# Autodesk Inventor assembly: platform
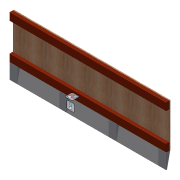
[picture p0: Inventor's stored thumbnail of the model, 180x180]
Saved by Autodesk Inventor 2015 (Build 190159000, 159)
## iProperties
Created: 2015-01-03
Part Number: platform
Document SubType Name: Assembly
Designer: Peter
Mass: 10587 g
Surface Area: 19021.5 cm^2
Volume: 16103.8 cm^3
Density: 0.657427 g/cm^3
Author: Peter
## Documents named in this file (5)
- T:\FILES\FIRST-Team-1719-CAD-Team\2015 Playing Field\Team 1719 Practice Field\Scoring Platform - Construction Design\platform.iam
- T:\FILES\FIRST-Team-1719-CAD-Team\2015 Playing Field\Team 1719 Practice Field\Scoring Platform - Construction Design\plywood platform.ipt
- T:\FILES\FIRST-Team-1719-CAD-Team\2015 Playing Field\Team 1719 Practice Field\Scoring Platform - Construction Design\2x4x48.ipt
- T:\FILES\FIRST-Team-1719-CAD-Team\2015 Playing Field\Team 1719 Practice Field\Scoring Platform - Construction Design\Ramp Assembly.iam
- T:\FILES\FIRST-Team-1719-CAD-Team\2015 Playing Field\Team 1719 Practice Field\Scoring Platform - Construction Design\Wedge.ipt
## Components (8 placed, 4 different names)
1. plywood platform:1 — Mate:1, Flush:1, Flush:2, Flush:3, Flush:4, Mate:2, Mate:3, Flush:5
2. 2x4x48:1 — Mate:1, Flush:1, Flush:2
3. 2x4x48:2 — Flush:3, Flush:4, Mate:2, Mate:4, Mate:5, Mate:6, Mate:7, Flush:6, Flush:7, Flush:8, Flush:9, Flush:10, Flush:11
4. Ramp Assembly:1 [sub-assembly] — Mate:3, Flush:5, Mate:10
5. Wedge:1 — Mate:6, Flush:8, Mate:8, Mate:9, Mate:10
6. Wedge:2 — Mate:4, Flush:6, Flush:10
7. Wedge:3 — Mate:5, Flush:7, Mate:9
8. Wedge:4 — Mate:7, Flush:9, Flush:11, Mate:8
## Relationships (21: Flush 11, Mate 10)
- Mate:1: plywood platform:1 ↔ 2x4x48:1
- Flush:1: plywood platform:1 ↔ 2x4x48:1
- Flush:2: plywood platform:1 ↔ 2x4x48:1
- Flush:3: plywood platform:1 ↔ 2x4x48:2
- Flush:4: plywood platform:1 ↔ 2x4x48:2
- Mate:2: plywood platform:1 ↔ 2x4x48:2
- Mate:3: plywood platform:1 ↔ Ramp Assembly:1
- Flush:5: plywood platform:1 ↔ Ramp Assembly:1
- Mate:4: 2x4x48:2 ↔ Wedge:2
- Mate:5: 2x4x48:2 ↔ Wedge:3
- Mate:6: 2x4x48:2 ↔ Wedge:1
- Mate:7: 2x4x48:2 ↔ Wedge:4
- Flush:6: 2x4x48:2 ↔ Wedge:2
- Flush:7: 2x4x48:2 ↔ Wedge:3
- Flush:8: 2x4x48:2 ↔ Wedge:1
- Flush:9: 2x4x48:2 ↔ Wedge:4
- Flush:10: 2x4x48:2 ↔ Wedge:2
- Flush:11: 2x4x48:2 ↔ Wedge:4
- Mate:8 (491.0667 mm): Wedge:1 ↔ Wedge:4
- Mate:9 (491.0667 mm): Wedge:1 ↔ Wedge:3
- Mate:10: Ramp Assembly:1 ↔ Wedge:1
